# Autodesk Inventor assembly: BGHK6800VV-20
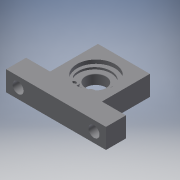
[picture p0: Inventor's stored thumbnail of the model, 180x180]
Saved by Autodesk Inventor 2019 (Build 230136000, 136)
## iProperties
Category: PARTsolutions
Company: MISUMI
Created: 2022-11-02
Part Number: BGHK6800VV-20
Catalog Web Link: www.cadenas.de
Description: BGHKB, BGHK, BGHKA, BGHKSA, BGHKS-Bearings with Housings T-Shaped h Selectable
Vendor: MISUMI
Document SubType Name: Assembly
Designer: psAdmin
Manufacturer: MISUMI
Mass: 9.17909 g
Surface Area: 56.1194 cm^2
Volume: 9.17909 cm^3
Density: 1 g/cm^3
Title: BGHK6800VV-20
Author: Cadenas PARTsolutions
Comments: Bearings with Housings T-Shaped h Selectable
PSOL_IDENT_0: {$CADENAS_DATA/23d-libs/misumi/metric/12_bearing_holders/bghkb_asmtab.prj},241 {VTYP=3D},{STYP=ASSTA
PSOL_IDENT_1: B},{NB=BGHK6800VV-20},{LINA=BGHK6800VV-20},{NN=BGHKB, BGHK, BGHKA, BGHKSA, BGHKS},{DATE=30.06.2021 1
PSOL_IDENT_2: 2:58:11},{GEOMDATE=09.07.2015 08:06:15},{VERSION=},{LINEID=300},{WBVAR=MATB,MATH,STH,SEAL,HH,ALT1,AL
PSOL_IDENT_3: T2},{WBNUMERIC=HH}  {NB=BGHK6800VV-20},{LINA=BGHK6800VV-20},{KT=DUMMY},{PN=BGHK6800VV-20},{TYPE=BGHK
PSOL_IDENT_4: },{MATB=S},{MATBALG='S','Steel','SS','Stainless Steel'},{MATH=S45C},{MATHALG='S45C','1045 Carbon Ste
PSOL_IDENT_5: el','2017AA','2017 Aluminum Alloy'},{STH=ENP},{STHALG='BO','Black Oxide','ENP','Electroless Nickel P
PSOL_IDENT_6: lating'},{ARR=304 Stainless Steel},{ARR3D=-S},{BN=6800},{SEAL=VV},{SEALALG='ZZ','Double Shielded','V
PSOL_IDENT_7: V','Non-Contact Sealed Rubber Seal','DD','Contact Sealed Rubber Seal'},{HH=20},{HHALG=[20,25,30]},{D
PSOL_IDENT_8: D=10},{D=19},{DD2=20},{MM=1.15},{DDHH=16},{B=5},{LL1=2},{H=34},{H2=14},{L=50},{L1=38.0},{L2=26},{T=1
PSOL_IDENT_9: 0},{S=10},{DD1=5.5},{ALT1=},{ALT2=},{PPATH=bghkb/bghkb_asmtpl.prj}
NB: BGHK6800VV-20
NN: BGHKB, BGHK, BGHKA, BGHKSA, BGHKS
NT: Bearings with Housings T-Shaped h Selectable
NBSYN: $PN.
LINA: BGHK6800VV-20
CATALOG: Misumi
PN: BGHK6800VV-20
MATB: Steel
MATH: 1045 Carbon Steel
STH: Electroless Nickel Plating
ARR: 304 Stainless Steel
BN: 6800
SEAL: Non-Contact Sealed Rubber Seal
HH: 20
DD: 10
D: 19
DDHH: 16
B: 5
LL1: 2
H: 34
L: 50
L1: 38
L2: 26
T: 10
S: 10
DD1: 5.5
ALT1: Bearings, Retaining Rings Assembled
ALT2: w/o KCC (C2 Chamfer)
SUPPLIER: MISUMI
ARTICLENO: BGHK6800VV-20
BOMINFO: BGHK6800VV-20
CREATOR: CADENAS GmbH
## Documents named in this file (4)
- e:\temp\worker_COMMON_6\temp\tmp_3884_44_KbP5p\format_0\BGHK6800VV-20.iam
- e:\temp\worker_COMMON_6\temp\tmp_3884_44_KbP5p\format_0\BGHK6800VV-20_h.ipt
- e:\temp\worker_COMMON_6\temp\tmp_3884_44_KbP5p\format_0\bearing_6800.ipt
- e:\temp\worker_COMMON_6\temp\tmp_3884_44_KbP5p\format_0\RRING-C-INT-S-19.ipt
## Components (3 placed, 3 different names)
1. BGHK6800VV-20_h:1 — to_bearing_XY@1 <-> to_housing_XY@2, to_bearing_Z@1 <-> to_housing_Z@2, to_bearing_YZ@1 <-> to_housing_YZ@2, to_rring_XY@1 <-> rr_XY@3, to_rring_Z@1 <-> rr_Z@3, to_rring_YZ@1 <-> rr_YZ@3
2. bearing_6800:1 — to_bearing_XY@1 <-> to_housing_XY@2, to_bearing_Z@1 <-> to_housing_Z@2, to_bearing_YZ@1 <-> to_housing_YZ@2
3. RRING-C-INT-S-19:1 — to_rring_XY@1 <-> rr_XY@3, to_rring_Z@1 <-> rr_Z@3, to_rring_YZ@1 <-> rr_YZ@3
## Relationships (6: Mate 4, Angle 2)
- to_bearing_XY@1 <-> to_housing_XY@2 [Mate]: BGHK6800VV-20_h:1 ↔ bearing_6800:1
- to_bearing_Z@1 <-> to_housing_Z@2 [Mate]: BGHK6800VV-20_h:1 ↔ bearing_6800:1
- to_bearing_YZ@1 <-> to_housing_YZ@2 [Angle] (0 deg): BGHK6800VV-20_h:1 ↔ bearing_6800:1
- to_rring_XY@1 <-> rr_XY@3 [Mate]: BGHK6800VV-20_h:1 ↔ RRING-C-INT-S-19:1
- to_rring_Z@1 <-> rr_Z@3 [Mate]: BGHK6800VV-20_h:1 ↔ RRING-C-INT-S-19:1
- to_rring_YZ@1 <-> rr_YZ@3 [Angle] (0 deg): BGHK6800VV-20_h:1 ↔ RRING-C-INT-S-19:1
